# Autodesk Inventor assembly: arm
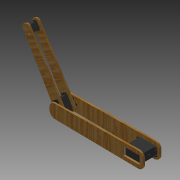
[picture p0: Inventor's stored thumbnail of the model, 180x180]
Saved by Autodesk Inventor 2013 (Build 170138000, 138)
## iProperties
Created: 2014-10-10
Part Number: arm
Document SubType Name: Assembly
Designer: Masta
Author: Masta
## Documents named in this file (3)
- D:\DrOctopus\3D model\arm.iam
- D:\DrOctopus\3D model\segment1.iam
- D:\DrOctopus\3D model\segment2.iam
## Components (2 placed, 2 different names)
1. segment1:1 [sub-assembly] — Insert:1
2. segment2:1 [sub-assembly] — Insert:1
## Relationships (1: Insert 1)
- Insert:1: segment1:1 ↔ segment2:1
